# Autodesk Inventor assembly: Chain Generator
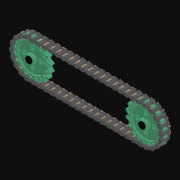
[picture p0: Inventor's stored thumbnail of the model, 180x180]
Saved by Autodesk Inventor 2021 (Build 250183000, 183)
## iProperties
Created: 2020-08-11
Part Number: Chain Generator
Document SubType Name: Assembly
Designer: yuany
Author: yuany
## Documents named in this file (10)
- E:\VEX Cad\Library 1.2\Motion\Chain Generator\Chain Generator.iam
- E:\VEX Cad\Library 1.2\Motion\Chain Generator\Pattern.ipt
- E:\VEX Cad\Library 1.2\Motion\Chain + Tank Tread\High Strength Chain Link.ipt
- E:\VEX Cad\Library 1.2\Motion\Sprockets\HS 18T Sprocket, Square.ipt
- E:\VEX Cad\Library 1.2\Motion\Chain + Tank Tread\Tank Tread Traction Link.ipt
- E:\VEX Cad\Library 1.2\Motion\Chain + Tank Tread\Tread Link.ipt
- E:\VEX Cad\Library 1.2\Motion\Chain + Tank Tread\Chain Attachment Link.ipt
- E:\VEX Cad\Library 1.2\Motion\Chain + Tank Tread\Short Flap.ipt
- E:\VEX Cad\Library 1.2\Motion\Chain + Tank Tread\Medium Flap.ipt
- E:\VEX Cad\Library 1.2\Motion\Chain + Tank Tread\Tall Flap.ipt
## Components (381 placed, 9 different names)
1. Pattern:1 — Mate:1, Angle:1, Mate:2, Mate:3, Insert:1, Angle:2, Insert:2, Angle:3, Mate:4, Mate:5, Angle:5, Mate:6, Angle:6, Mate:7, Angle:7, Mate:8, Angle:8, Mate:9, Angle:9
2. HS 18T Sprocket, Square:1 — Insert:1, Angle:2
3. HS 18T Sprocket, Square:2 — Insert:2, Angle:3
4. High Strength Chain Link:1 — Mate:1, Angle:1, Mate:2, Mate:3, Angle:4, Flush:1
5. High Strength Chain Link:2
6. High Strength Chain Link:3
7. High Strength Chain Link:4
8. High Strength Chain Link:5
9. High Strength Chain Link:6
10. High Strength Chain Link:7
11. High Strength Chain Link:8
12. High Strength Chain Link:9
13. High Strength Chain Link:10
14. High Strength Chain Link:11
15. High Strength Chain Link:12
16. High Strength Chain Link:13
17. High Strength Chain Link:14
18. High Strength Chain Link:15
19. High Strength Chain Link:16
20. High Strength Chain Link:17
21. High Strength Chain Link:18
22. High Strength Chain Link:19
23. High Strength Chain Link:20
24. High Strength Chain Link:21
25. High Strength Chain Link:22
26. High Strength Chain Link:23
27. High Strength Chain Link:24
28. High Strength Chain Link:25
29. High Strength Chain Link:26
30. High Strength Chain Link:27
31. High Strength Chain Link:28
32. High Strength Chain Link:29
33. High Strength Chain Link:30
34. High Strength Chain Link:31
35. High Strength Chain Link:32
36. High Strength Chain Link:33
37. High Strength Chain Link:34
38. High Strength Chain Link:35
39. High Strength Chain Link:36
40. High Strength Chain Link:37
41. High Strength Chain Link:38
42. High Strength Chain Link:39
43. High Strength Chain Link:40
44. High Strength Chain Link:41
45. High Strength Chain Link:42
46. High Strength Chain Link:43
47. High Strength Chain Link:44
48. High Strength Chain Link:45
49. High Strength Chain Link:46
50. High Strength Chain Link:47
51. High Strength Chain Link:48
52. High Strength Chain Link:49
53. High Strength Chain Link:50
54. High Strength Chain Link:51
55. High Strength Chain Link:52
56. High Strength Chain Link:53
57. High Strength Chain Link:54
58. Tank Tread Traction Link:1 — Angle:4, Mate:4, Flush:1, Flush:2
59. Tank Tread Traction Link:2
60. Tank Tread Traction Link:3
61. Tank Tread Traction Link:4
62. Tank Tread Traction Link:5
63. Tank Tread Traction Link:6
64. Tank Tread Traction Link:7
65. Tank Tread Traction Link:8
66. Tank Tread Traction Link:9
67. Tank Tread Traction Link:10
68. Tank Tread Traction Link:11
69. Tank Tread Traction Link:12
70. Tank Tread Traction Link:13
71. Tank Tread Traction Link:14
72. Tank Tread Traction Link:15
73. Tank Tread Traction Link:16
74. Tank Tread Traction Link:17
75. Tank Tread Traction Link:18
76. Tank Tread Traction Link:19
77. Tank Tread Traction Link:20
78. Tank Tread Traction Link:21
79. Tank Tread Traction Link:22
80. Tank Tread Traction Link:23
81. Tank Tread Traction Link:24
82. Tank Tread Traction Link:25
83. Tank Tread Traction Link:26
84. Tank Tread Traction Link:27
85. Tank Tread Traction Link:28
86. Tank Tread Traction Link:29
87. Tank Tread Traction Link:30
88. Tank Tread Traction Link:31
89. Tank Tread Traction Link:32
90. Tank Tread Traction Link:33
91. Tank Tread Traction Link:34
92. Tank Tread Traction Link:35
93. Tank Tread Traction Link:36
94. Tank Tread Traction Link:37
95. Tank Tread Traction Link:38
96. Tank Tread Traction Link:39
97. Tank Tread Traction Link:40
98. Tank Tread Traction Link:41
99. Tank Tread Traction Link:42
100. Tank Tread Traction Link:43
101. Tank Tread Traction Link:44
102. Tank Tread Traction Link:45
103. Tank Tread Traction Link:46
104. Tank Tread Traction Link:47
105. Tank Tread Traction Link:48
106. Tank Tread Traction Link:49
107. Tank Tread Traction Link:50
108. Tank Tread Traction Link:51
109. Tank Tread Traction Link:52
110. Tank Tread Traction Link:53
111. Tank Tread Traction Link:54
112. Tread Link:1 — Flush:2, Mate:5, Angle:5, Flush:3
113. Tread Link:2
114. Tread Link:3
115. Tread Link:4
116. Tread Link:5
117. Tread Link:6
118. Tread Link:7
119. Tread Link:8
120. Tread Link:9
121. Tread Link:10
122. Tread Link:11
123. Tread Link:12
124. Tread Link:13
125. Tread Link:14
126. Tread Link:15
127. Tread Link:16
128. Tread Link:17
129. Tread Link:18
130. Tread Link:19
131. Tread Link:20
132. Tread Link:21
133. Tread Link:22
134. Tread Link:23
135. Tread Link:24
136. Tread Link:25
137. Tread Link:26
138. Tread Link:27
139. Tread Link:28
140. Tread Link:29
141. Tread Link:30
142. Tread Link:31
143. Tread Link:32
144. Tread Link:33
145. Tread Link:34
146. Tread Link:35
147. Tread Link:36
148. Tread Link:37
149. Tread Link:38
150. Tread Link:39
151. Tread Link:40
152. Tread Link:41
153. Tread Link:42
154. Tread Link:43
155. Tread Link:44
156. Tread Link:45
157. Tread Link:46
158. Tread Link:47
159. Tread Link:48
160. Tread Link:49
161. Tread Link:50
162. Tread Link:51
163. Tread Link:52
164. Tread Link:53
165. Tread Link:54
166. Chain Attachment Link:1 — Mate:6, Flush:3, Angle:6, Flush:4
167. Chain Attachment Link:2
168. Chain Attachment Link:3
169. Chain Attachment Link:4
170. Chain Attachment Link:5
171. Chain Attachment Link:6
172. Chain Attachment Link:7
173. Chain Attachment Link:8
174. Chain Attachment Link:9
175. Chain Attachment Link:10
176. Chain Attachment Link:11
177. Chain Attachment Link:12
178. Chain Attachment Link:13
179. Chain Attachment Link:14
180. Chain Attachment Link:15
181. Chain Attachment Link:16
182. Chain Attachment Link:17
183. Chain Attachment Link:18
184. Chain Attachment Link:19
185. Chain Attachment Link:20
186. Chain Attachment Link:21
187. Chain Attachment Link:22
188. Chain Attachment Link:23
189. Chain Attachment Link:24
190. Chain Attachment Link:25
191. Chain Attachment Link:26
192. Chain Attachment Link:27
193. Chain Attachment Link:28
194. Chain Attachment Link:29
195. Chain Attachment Link:30
196. Chain Attachment Link:31
197. Chain Attachment Link:32
198. Chain Attachment Link:33
199. Chain Attachment Link:34
200. Chain Attachment Link:35
201. Chain Attachment Link:36
202. Chain Attachment Link:37
203. Chain Attachment Link:38
204. Chain Attachment Link:39
205. Chain Attachment Link:40
206. Chain Attachment Link:41
207. Chain Attachment Link:42
208. Chain Attachment Link:43
209. Chain Attachment Link:44
210. Chain Attachment Link:45
211. Chain Attachment Link:46
212. Chain Attachment Link:47
213. Chain Attachment Link:48
214. Chain Attachment Link:49
215. Chain Attachment Link:50
216. Chain Attachment Link:51
217. Chain Attachment Link:52
218. Chain Attachment Link:53
219. Chain Attachment Link:54
220. Short Flap:1 — Mate:7, Flush:4, Angle:7, Flush:5
221. Short Flap:2
222. Short Flap:3
223. Short Flap:4
224. Short Flap:5
225. Short Flap:6
226. Short Flap:7
227. Short Flap:8
228. Short Flap:9
229. Short Flap:10
230. Short Flap:11
231. Short Flap:12
232. Short Flap:13
233. Short Flap:14
234. Short Flap:15
235. Short Flap:16
236. Short Flap:17
237. Short Flap:18
238. Short Flap:19
239. Short Flap:20
240. Short Flap:21
241. Short Flap:22
242. Short Flap:23
243. Short Flap:24
244. Short Flap:25
245. Short Flap:26
246. Short Flap:27
247. Short Flap:28
248. Short Flap:29
249. Short Flap:30
250. Short Flap:31
251. Short Flap:32
252. Short Flap:33
253. Short Flap:34
254. Short Flap:35
255. Short Flap:36
256. Short Flap:37
257. Short Flap:38
258. Short Flap:39
259. Short Flap:40
260. Short Flap:41
261. Short Flap:42
262. Short Flap:43
263. Short Flap:44
264. Short Flap:45
265. Short Flap:46
266. Short Flap:47
267. Short Flap:48
268. Short Flap:49
269. Short Flap:50
270. Short Flap:51
271. Short Flap:52
272. Short Flap:53
273. Short Flap:54
274. Medium Flap:1 — Mate:8, Flush:5, Angle:8, Flush:6
275. Medium Flap:2
276. Medium Flap:3
277. Medium Flap:4
278. Medium Flap:5
279. Medium Flap:6
280. Medium Flap:7
281. Medium Flap:8
282. Medium Flap:9
283. Medium Flap:10
284. Medium Flap:11
285. Medium Flap:12
286. Medium Flap:13
287. Medium Flap:14
288. Medium Flap:15
289. Medium Flap:16
290. Medium Flap:17
291. Medium Flap:18
292. Medium Flap:19
293. Medium Flap:20
294. Medium Flap:21
295. Medium Flap:22
296. Medium Flap:23
297. Medium Flap:24
298. Medium Flap:25
299. Medium Flap:26
300. Medium Flap:27
301. Medium Flap:28
302. Medium Flap:29
303. Medium Flap:30
304. Medium Flap:31
305. Medium Flap:32
306. Medium Flap:33
307. Medium Flap:34
308. Medium Flap:35
309. Medium Flap:36
310. Medium Flap:37
311. Medium Flap:38
312. Medium Flap:39
313. Medium Flap:40
314. Medium Flap:41
315. Medium Flap:42
316. Medium Flap:43
317. Medium Flap:44
318. Medium Flap:45
319. Medium Flap:46
320. Medium Flap:47
321. Medium Flap:48
322. Medium Flap:49
323. Medium Flap:50
324. Medium Flap:51
325. Medium Flap:52
326. Medium Flap:53
327. Medium Flap:54
328. Tall Flap:1 — Flush:6, Mate:9, Angle:9
329. Tall Flap:2
330. Tall Flap:3
331. Tall Flap:4
332. Tall Flap:5
333. Tall Flap:6
334. Tall Flap:7
335. Tall Flap:8
336. Tall Flap:9
337. Tall Flap:10
338. Tall Flap:11
339. Tall Flap:12
340. Tall Flap:13
341. Tall Flap:14
342. Tall Flap:15
343. Tall Flap:16
344. Tall Flap:17
345. Tall Flap:18
346. Tall Flap:19
347. Tall Flap:20
348. Tall Flap:21
349. Tall Flap:22
350. Tall Flap:23
351. Tall Flap:24
352. Tall Flap:25
353. Tall Flap:26
354. Tall Flap:27
355. Tall Flap:28
356. Tall Flap:29
357. Tall Flap:30
358. Tall Flap:31
359. Tall Flap:32
360. Tall Flap:33
361. Tall Flap:34
362. Tall Flap:35
363. Tall Flap:36
364. Tall Flap:37
365. Tall Flap:38
366. Tall Flap:39
367. Tall Flap:40
368. Tall Flap:41
369. Tall Flap:42
370. Tall Flap:43
371. Tall Flap:44
372. Tall Flap:45
373. Tall Flap:46
374. Tall Flap:47
375. Tall Flap:48
376. Tall Flap:49
377. Tall Flap:50
378. Tall Flap:51
379. Tall Flap:52
380. Tall Flap:53
381. Tall Flap:54
## Component patterns: Chain (54 elements), Traction (54 elements), Tread (54 elements), Chain Attachment (54 elements), Short Flaps (54 elements), Medium Flaps (54 elements), Tall Flaps (54 elements)
## Relationships (26: Mate 9, Angle 9, Flush 6, Insert 2)
- Mate:1: Pattern:1 ↔ High Strength Chain Link:1
- Angle:1 (-90 deg): Pattern:1 ↔ High Strength Chain Link:1
- Mate:2: Pattern:1 ↔ High Strength Chain Link:1
- Mate:3 (0.8387 mm): Pattern:1 ↔ High Strength Chain Link:1
- Insert:1: Pattern:1 ↔ HS 18T Sprocket, Square:1
- Angle:2 (90 deg): Pattern:1 ↔ HS 18T Sprocket, Square:1
- Insert:2: Pattern:1 ↔ HS 18T Sprocket, Square:2
- Angle:3 (90 deg): Pattern:1 ↔ HS 18T Sprocket, Square:2
- Angle:4 (180 deg): High Strength Chain Link:1 ↔ Tank Tread Traction Link:1
- Mate:4: Pattern:1 ↔ Tank Tread Traction Link:1
- Flush:1: High Strength Chain Link:1 ↔ Tank Tread Traction Link:1
- Flush:2: Tank Tread Traction Link:1 ↔ Tread Link:1
- Mate:5: Pattern:1 ↔ Tread Link:1
- Angle:5 (90 deg): Pattern:1 ↔ Tread Link:1
- Mate:6: Pattern:1 ↔ Chain Attachment Link:1
- Flush:3: Tread Link:1 ↔ Chain Attachment Link:1
- Angle:6 (90 deg): Pattern:1 ↔ Chain Attachment Link:1
- Mate:7: Pattern:1 ↔ Short Flap:1
- Flush:4: Chain Attachment Link:1 ↔ Short Flap:1
- Angle:7 (-90 deg): Pattern:1 ↔ Short Flap:1
- Mate:8: Pattern:1 ↔ Medium Flap:1
- Flush:5: Short Flap:1 ↔ Medium Flap:1
- Angle:8 (-90 deg): Pattern:1 ↔ Medium Flap:1
- Flush:6: Medium Flap:1 ↔ Tall Flap:1
- Mate:9: Pattern:1 ↔ Tall Flap:1
- Angle:9 (90 deg): Pattern:1 ↔ Tall Flap:1
## Named parameters: Sprocket2Angle = 90 deg, CenterDistance = 177.8 mm, Sprocket1 = 56.388 mm, Sprocket2 = 56.388 mm, CurveLength = 532.74813 mm, Center_Distance = 177.8 mm
